# Autodesk Inventor assembly: gusset_mirrored
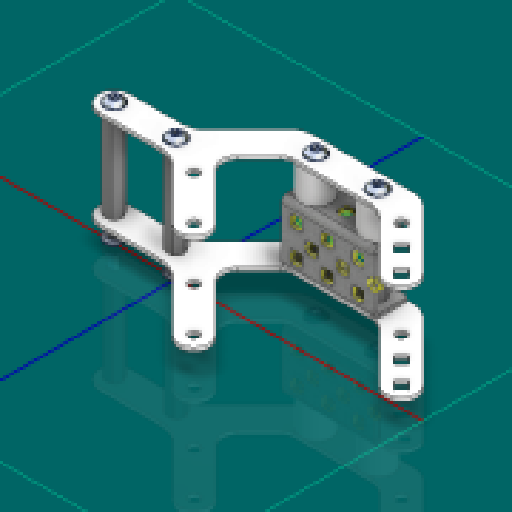
[picture p0: Inventor's stored thumbnail of the model, 512x512]
Saved by Autodesk Inventor 2025 (Build 290162000, 162)
## iProperties
Created: 2024-08-17
Part Number: gusset_mirrored
Document SubType Name: Assembly
Designer: averey
Author: averey
## Documents named in this file (11)
- C:\Users\avere\vex_robotics_high_stakes\hardware\cad\ATLAS\chassis\drive_pod\gusset_mirrored\gusset_mirrored.iam
- C:\Users\avere\vex_robotics_high_stakes\hardware\cad\ATLAS\chassis\drive_pod\gusset_mirrored\join_gusset_mirrored.ipt
- C:\Users\avere\vex_robotics_high_stakes\hardware\cad\VEX-CAD-Inventor\Motion\Spacers\Spacer Nylon .500 OD\NSpacer White .500 OD x .500.ipt
- C:\Users\avere\vex_robotics_high_stakes\hardware\cad\VEX-CAD-Inventor\Motion\Spacers\Spacer Nylon .500 OD.ipt
- C:\Users\avere\vex_robotics_high_stakes\hardware\cad\ATLAS\chassis\drive_pod\gusset_mirrored\Alu C 1x2x1x3_mirrored.ipt
- C:\Users\avere\vex_robotics_high_stakes\hardware\cad\VEX-CAD-Inventor\Structure\Standoff\Standoff .875.ipt
- C:\Users\avere\vex_robotics_high_stakes\hardware\cad\VEX-CAD-Inventor\Structure\Standoff.ipt
- C:\Users\avere\vex_robotics_high_stakes\hardware\cad\VEX-CAD-Inventor\Structure\Hardware\Screw Steel - Star\SScrew Star Smooth .750.ipt
- C:\Users\avere\vex_robotics_high_stakes\hardware\cad\VEX-CAD-Inventor\Structure\Hardware\Screw Steel - Star.ipt
- C:\Users\avere\vex_robotics_high_stakes\hardware\cad\VEX-CAD-Inventor\Structure\Hardware\Screw Shoulder Robosource\SScrew Shoulder Smooth .375 x .12.ipt
- C:\Users\avere\vex_robotics_high_stakes\hardware\cad\VEX-CAD-Inventor\Structure\Hardware\Screw Shoulder Robosource.ipt
## Components (15 placed, 6 different names)
1. join_gusset_mirrored:1 — Mate:1, Insert:1, Insert:15, Insert:17
2. join_gusset_mirrored:2 — Mate:1, Insert:1, Insert:5, Insert:7, Insert:14, Insert:13, Insert:23, Insert:21, Insert:21, Insert:22
3. NSpacer White .500 OD x .500:1 — Insert:5, Insert:8
4. NSpacer White .500 OD x .500:2 — Insert:7, Mate:2
5. Alu C 1x2x1x3_mirrored:1 — Mate:2, Insert:8, Insert:9, Insert:10
6. Standoff .875:1 — Insert:9
7. Standoff .875:2 — Insert:10
8. SScrew Star Smooth .750:1 — Insert:14
9. SScrew Star Smooth .750:2 — Insert:13
10. SScrew Shoulder Smooth .375 x .12:1 — Insert:15
11. SScrew Shoulder Smooth .375 x .12:2 — Insert:17
12. SScrew Star Smooth .750:4 — Insert:23
13. SScrew Star Smooth .750:6 — Insert:21
14. NSpacer White .500 OD x .500:3 — Insert:22
15. NSpacer White .500 OD x .500:4 — Insert:21
## Relationships (16: Insert 14, Mate 2)
- Mate:1: join_gusset_mirrored:1 ↔ join_gusset_mirrored:2
- Insert:1 (38.1 mm): join_gusset_mirrored:1 ↔ join_gusset_mirrored:2
- Insert:5: join_gusset_mirrored:2 ↔ NSpacer White .500 OD x .500:1
- Insert:7: join_gusset_mirrored:2 ↔ NSpacer White .500 OD x .500:2
- Mate:2: NSpacer White .500 OD x .500:2 ↔ Alu C 1x2x1x3_mirrored:1
- Insert:8: NSpacer White .500 OD x .500:1 ↔ Alu C 1x2x1x3_mirrored:1
- Insert:9: Alu C 1x2x1x3_mirrored:1 ↔ Standoff .875:1
- Insert:10: Alu C 1x2x1x3_mirrored:1 ↔ Standoff .875:2
- Insert:14: join_gusset_mirrored:2 ↔ SScrew Star Smooth .750:1
- Insert:13: join_gusset_mirrored:2 ↔ SScrew Star Smooth .750:2
- Insert:15: join_gusset_mirrored:1 ↔ SScrew Shoulder Smooth .375 x .12:1
- Insert:17: join_gusset_mirrored:1 ↔ SScrew Shoulder Smooth .375 x .12:2
- Insert:23: join_gusset_mirrored:2 ↔ SScrew Star Smooth .750:4
- Insert:21: join_gusset_mirrored:2 ↔ SScrew Star Smooth .750:6
- Insert:21: join_gusset_mirrored:2 ↔ NSpacer White .500 OD x .500:4
- Insert:22: join_gusset_mirrored:2 ↔ NSpacer White .500 OD x .500:3
